# Autodesk Inventor assembly: LearningKitPotiBox
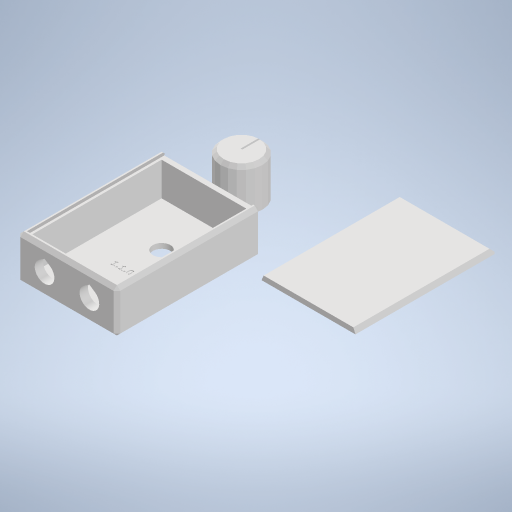
[picture p0: Inventor's stored thumbnail of the model, 512x512]
Saved by Autodesk Inventor 2024.3 (Build 283343000, 343)
## iProperties
Created: 2025-03-30
Part Number: LearningKitPotiBox
Document SubType Name: Assembly
Designer: maxho
Author: maxho
## Documents named in this file (4)
- Z:\Dokumente\LearningKit\LearningKitPotiBox\LearningKitPotiBox.iam
- Z:\Dokumente\LearningKit\LearningKitPotiBox\PotiBoxCase.ipt
- Z:\Dokumente\LearningKit\LearningKitPotiBox\PotiBoxKnob.ipt
- Z:\Dokumente\LearningKit\LearningKitPotiBox\PotiBoxLid.ipt
## Components (3 placed, 3 different names)
1. PotiBoxCase:1 — Passend:1, Passend:2, Passend:3
2. PotiBoxKnob:1
3. PotiBoxLid:1
## Relationships (3: Mate 3)
- Passend:1 [Mate]: PotiBoxCase:1
- Passend:2 [Mate]: PotiBoxCase:1
- Passend:3 [Mate]: PotiBoxCase:1
